# Autodesk Inventor assembly: Stand
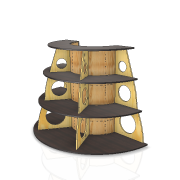
[picture p0: Inventor's stored thumbnail of the model, 180x180]
Saved by Autodesk Inventor 2024.3 (Build 283343000, 343)
## iProperties
Created: 2020-04-20
Part Number: Stand
Document SubType Name: Assembly
Designer: SauliusD
Author: SauliusD
## Documents named in this file (17)
- C:\W4INV 2024 Design\PROJECTS\Samples\Stand\Stand.iam
- C:\W4INV 2024 Design\PROJECTS\Samples\Stand\Right Strut.ipt
- C:\W4INV 2024 Design\PROJECTS\Samples\Stand\Left Strut.ipt
- C:\W4INV 2024 Design\PROJECTS\Samples\Stand\Middle Right Strut.ipt
- C:\W4INV 2024 Design\PROJECTS\Samples\Stand\Miffle Left Strut.ipt
- C:\W4INV 2024 Design\PROJECTS\Samples\Stand\Bootom.ipt
- C:\W4INV 2024 Design\PROJECTS\Samples\Stand\Top.ipt
- C:\W4INV 2024 Design\PROJECTS\Samples\Stand\Lower Shelf.ipt
- C:\W4INV 2024 Design\PROJECTS\Samples\Stand\Upper Shelf.ipt
- C:\W4INV 2024 Design\PROJECTS\Samples\Stand\Back.ipt
- C:\W4INV 2024 Design\_LIBRARY\Fixed joints\Minifix joint\MINIFIX D15 v2\Minifix D15 & Dowel L34 & Cap D15 PB T18 LH.ipt
- C:\W4INV 2024 Design\_LIBRARY\Fixed joints\Minifix joint\MINIFIX D15 v2\Minifix D15 & Dowel L34 & Cap D15 PB T18 RH.ipt
- C:\W4INV 2024 Design\_LIBRARY\Fixed joints\Confirmat\CONFIRMAT\Confirmat L50 & Cap D10 NB T18 PB T 18.ipt
- C:\W4INV 2024 Design\_LIBRARY\Supports and legs\Supports\ADJUSTABLE SUPPORT\Support M6 H27 D18 with Bushing SB T18.ipt
- C:\W4INV 2024 Design\LIBRARY\Fixed joints\Confirmat\CONFIRMAT.ipt
- C:\W4INV 2024 Design\LIBRARY\Fixed joints\Minifix joint\MINIFIX D15 v2.ipt
- C:\W4INV 2024 Design\LIBRARY\Supports and legs\Supports\ADJUSTABLE SUPPORT.ipt
## Components (37 placed, 13 different names)
1. Right Strut:1 — Flush:1, Pillar Board Side Plane :1, Pillar Board Side Plane :2, Pillar Board Side Plane:1, Pillar Board Side Plane:2, Pillar Board Side Plane:3, Nestled Board Plane:6, Nestled Board Plane:7, Nestled Board Plane:8, Side board:1, Side board:2
2. Left Strut:1 — Pillar Board Side Plane :3, Pillar Board Side Plane :4
3. Middle Right Strut:1
4. Miffle Left Strut:1
5. Bootom:1 — Nestled Board Plane:3, Nestled Board Plane:4, Nestled Board Plane:5, Bottom board:1, Bottom board:2
6. Top:1 — Nestled Board Plane:1, Nestled Board Plane:2, Nestled Board Plane:9, Nestled Board Plane:10
7. Lower Shelf:1 — Pillar Board Side Plane:6
8. Upper Shelf:1 — Pillar Board Side Plane:4, Pillar Board Side Plane:5
9. Back:1
10. Minifix D15 & Dowel L34 & Cap D15 PB T18 RH:1 — Axis Plane:1, Nestled Board Plane:1, Pillar Board Side Plane :1
11. Minifix D15 & Dowel L34 & Cap D15 PB T18 LH:2 — Axis Plane:2, Nestled Board Plane:2, Pillar Board Side Plane :2
12. Confirmat L50 & Cap D10 NB T18 PB T 18:10 — Mate:13
13. Confirmat L50 & Cap D10 NB T18 PB T 18:11 — Mate:14
14. Confirmat L50 & Cap D10 NB T18 PB T 18:12 — Mate:15
15. Confirmat L50 & Cap D10 NB T18 PB T 18:13 — Axis Plane:6, Nestled Board Plane:6, Pillar Board Side Plane:4
16. Confirmat L50 & Cap D10 NB T18 PB T 18:14 — Axis Plane:7, Nestled Board Plane:7, Pillar Board Side Plane:5
17. Confirmat L50 & Cap D10 NB T18 PB T 18:15 — Nestled Board Plane:8, Pillar Board Side Plane:6, Axis Plane:8
18. Confirmat L50 & Cap D10 NB T18 PB T 18:16 — Mate:22
19. Support M6 H27 D18 with Bushing SB T18:7 — Mate:27
20. Support M6 H27 D18 with Bushing SB T18:8 — Mate:28
21. Minifix D15 & Dowel L34 & Cap D15 PB T18 LH:3 — Axis Plane:9, Nestled Board Plane:9, Pillar Board Side Plane :3
22. Minifix D15 & Dowel L34 & Cap D15 PB T18 RH:4 — Axis Plane:10, Nestled Board Plane:10, Pillar Board Side Plane :4
23. Confirmat L50 & Cap D10 NB T18 PB T 18:1 — Axis Plane:3, Nestled Board Plane:3, Pillar Board Side Plane:1
24. Confirmat L50 & Cap D10 NB T18 PB T 18:2 — Axis Plane:4, Nestled Board Plane:4, Pillar Board Side Plane:2
25. Confirmat L50 & Cap D10 NB T18 PB T 18:3 — Axis Plane:5, Nestled Board Plane:5, Pillar Board Side Plane:3
26. Confirmat L50 & Cap D10 NB T18 PB T 18:4
27. Confirmat L50 & Cap D10 NB T18 PB T 18:5
28. Confirmat L50 & Cap D10 NB T18 PB T 18:6
29. Confirmat L50 & Cap D10 NB T18 PB T 18:7
30. Confirmat L50 & Cap D10 NB T18 PB T 18:8
31. Confirmat L50 & Cap D10 NB T18 PB T 18:9
32. Support M6 H27 D18 with Bushing SB T18:1 — Axis:1, Bottom board:1, Side board:1
33. Support M6 H27 D18 with Bushing SB T18:2 — Axis:2, Bottom board:2, Side board:2
34. Support M6 H27 D18 with Bushing SB T18:3
35. Support M6 H27 D18 with Bushing SB T18:4
36. Support M6 H27 D18 with Bushing SB T18:5
37. Support M6 H27 D18 with Bushing SB T18:6
## Component patterns: (3 elements, first: Confirmat L50 & Cap D10 NB T18 PB T 18:1 + Confirmat L50 & Cap D10 NB T18 PB T 18:2 + Confirmat L50 & Cap D10 NB T18 PB T 18:3), (3 elements, first: Support M6 H27 D18 with Bushing SB T18:1 + Support M6 H27 D18 with Bushing SB T18:2)
## Relationships (52: Mate 30, Flush 22)
- Flush:1 (-30 mm): Right Strut:1
- Flush:2 (-120 mm)
- Axis Plane:1 [Mate]: Minifix D15 & Dowel L34 & Cap D15 PB T18 RH:1
- Nestled Board Plane:1 [Mate]: Top:1 ↔ Minifix D15 & Dowel L34 & Cap D15 PB T18 RH:1
- Pillar Board Side Plane :1 [Flush] (18 mm): Right Strut:1 ↔ Minifix D15 & Dowel L34 & Cap D15 PB T18 RH:1
- Axis Plane:2 [Mate]: Minifix D15 & Dowel L34 & Cap D15 PB T18 LH:2
- Nestled Board Plane:2 [Mate]: Top:1 ↔ Minifix D15 & Dowel L34 & Cap D15 PB T18 LH:2
- Pillar Board Side Plane :2 [Flush] (18 mm): Right Strut:1 ↔ Minifix D15 & Dowel L34 & Cap D15 PB T18 LH:2
- Flush:5 (-120 mm)
- Flush:6 (-432 mm)
- Axis Plane:3 [Mate]: Confirmat L50 & Cap D10 NB T18 PB T 18:1
- Nestled Board Plane:3 [Flush]: Bootom:1 ↔ Confirmat L50 & Cap D10 NB T18 PB T 18:1
- Pillar Board Side Plane:1 [Mate] (-9 mm): Right Strut:1 ↔ Confirmat L50 & Cap D10 NB T18 PB T 18:1
- Axis Plane:4 [Mate]: Confirmat L50 & Cap D10 NB T18 PB T 18:2
- Nestled Board Plane:4 [Flush]: Bootom:1 ↔ Confirmat L50 & Cap D10 NB T18 PB T 18:2
- Pillar Board Side Plane:2 [Mate] (-9 mm): Right Strut:1 ↔ Confirmat L50 & Cap D10 NB T18 PB T 18:2
- Axis Plane:5 [Mate]: Confirmat L50 & Cap D10 NB T18 PB T 18:3
- Nestled Board Plane:5 [Flush]: Bootom:1 ↔ Confirmat L50 & Cap D10 NB T18 PB T 18:3
- Pillar Board Side Plane:3 [Mate] (-9 mm): Right Strut:1 ↔ Confirmat L50 & Cap D10 NB T18 PB T 18:3
- Flush:10 (-120 mm)
- Flush:11 (-432 mm)
- Mate:13: Confirmat L50 & Cap D10 NB T18 PB T 18:10
- Mate:14: Confirmat L50 & Cap D10 NB T18 PB T 18:11
- Mate:15: Confirmat L50 & Cap D10 NB T18 PB T 18:12
- Axis Plane:6 [Mate]: Confirmat L50 & Cap D10 NB T18 PB T 18:13
- Nestled Board Plane:6 [Flush]: Right Strut:1 ↔ Confirmat L50 & Cap D10 NB T18 PB T 18:13
- Pillar Board Side Plane:4 [Mate] (-9 mm): Upper Shelf:1 ↔ Confirmat L50 & Cap D10 NB T18 PB T 18:13
- Axis Plane:7 [Mate]: Confirmat L50 & Cap D10 NB T18 PB T 18:14
- Nestled Board Plane:7 [Flush]: Right Strut:1 ↔ Confirmat L50 & Cap D10 NB T18 PB T 18:14
- Pillar Board Side Plane:5 [Mate] (-9 mm): Upper Shelf:1 ↔ Confirmat L50 & Cap D10 NB T18 PB T 18:14
- Flush:14 (-132 mm)
- Nestled Board Plane:8 [Flush]: Right Strut:1 ↔ Confirmat L50 & Cap D10 NB T18 PB T 18:15
- Pillar Board Side Plane:6 [Mate] (-9 mm): Lower Shelf:1 ↔ Confirmat L50 & Cap D10 NB T18 PB T 18:15
- Axis Plane:8 [Mate]: Confirmat L50 & Cap D10 NB T18 PB T 18:15
- Mate:22: Confirmat L50 & Cap D10 NB T18 PB T 18:16
- Flush:16 (-20 mm)
- Flush:17 (-40 mm)
- Axis:1 [Mate]: Support M6 H27 D18 with Bushing SB T18:1
- Bottom board:1 [Mate] (17.5 mm): Bootom:1 ↔ Support M6 H27 D18 with Bushing SB T18:1
- Side board:1 [Flush] (9 mm): Right Strut:1 ↔ Support M6 H27 D18 with Bushing SB T18:1
- Axis:2 [Mate]: Support M6 H27 D18 with Bushing SB T18:2
- Bottom board:2 [Mate] (17.5 mm): Bootom:1 ↔ Support M6 H27 D18 with Bushing SB T18:2
- Side board:2 [Flush] (9 mm): Right Strut:1 ↔ Support M6 H27 D18 with Bushing SB T18:2
- Mate:27: Support M6 H27 D18 with Bushing SB T18:7
- Mate:28: Support M6 H27 D18 with Bushing SB T18:8
- Flush:20 (-120 mm)
- Axis Plane:9 [Mate]: Minifix D15 & Dowel L34 & Cap D15 PB T18 LH:3
- Nestled Board Plane:9 [Mate]: Top:1 ↔ Minifix D15 & Dowel L34 & Cap D15 PB T18 LH:3
- Pillar Board Side Plane :3 [Flush] (18 mm): Left Strut:1 ↔ Minifix D15 & Dowel L34 & Cap D15 PB T18 LH:3
- Axis Plane:10 [Mate]: Minifix D15 & Dowel L34 & Cap D15 PB T18 RH:4
- Nestled Board Plane:10 [Mate]: Top:1 ↔ Minifix D15 & Dowel L34 & Cap D15 PB T18 RH:4
- Pillar Board Side Plane :4 [Flush] (18 mm): Left Strut:1 ↔ Minifix D15 & Dowel L34 & Cap D15 PB T18 RH:4
